# Autodesk Inventor assembly: Assembly1
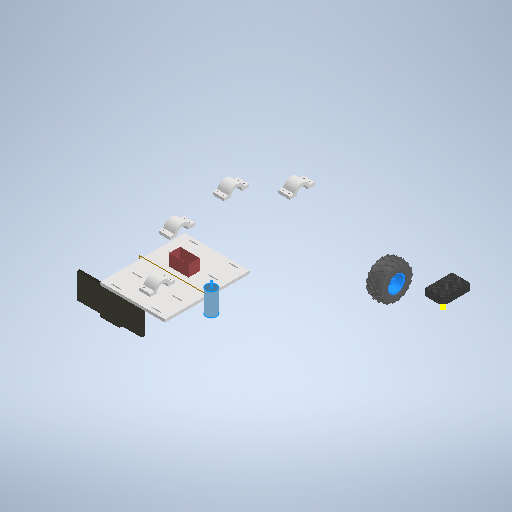
[picture p0: Inventor's stored thumbnail of the model, 512x512]
Saved by Autodesk Inventor 2025.3 (Build 293356030, 356C)
## iProperties
Created: 2026-06-25
Part Number: Assembly1
Document SubType Name: Assembly
Designer: user
Author: user
## Documents named in this file (8)
- C:\Docs\shcool\dojo\Design_\Assembly1.iam
- C:\Docs\shcool\dojo\Design_\base.ipt
- C:\Docs\shcool\dojo\Design_\front.ipt
- C:\Docs\shcool\dojo\Design_\motor.ipt
- C:\Docs\shcool\dojo\Design_\pi.ipt
- C:\Docs\shcool\dojo\Design_\Spiked Rubber Wheel 120mm.ipt
- C:\Docs\shcool\dojo\Design_\U_bracket.ipt
- C:\Docs\shcool\dojo\Design_\batteries.ipt
## Components (10 placed, 7 different names)
1. base:1 — Symmetry:1
2. front:1
3. motor:1
4. pi:1
5. Spiked Rubber Wheel 120mm:1
6. U_bracket:1
7. U_bracket:2
8. U_bracket:3
9. U_bracket:4
10. batteries:1
## Relationships (1: Symmetry 1)
- Symmetry:1: base:1
